# Autodesk Inventor assembly: RobotTable
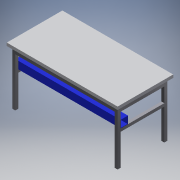
[picture p0: Inventor's stored thumbnail of the model, 180x180]
Saved by Autodesk Inventor 2017 (Build 210142000, 142)
## iProperties
Created: 2018-08-24
Part Number: RobotTable
Document SubType Name: Assembly
Designer: emmacarlisle
Author: emmacarlisle
## Documents named in this file (4)
- \\Mac\Home\Documents\RobotTable.iam
- \\Mac\Home\Documents\bottomtable.ipt
- \\Mac\Home\Documents\toptable.ipt
- \\Mac\Home\Documents\bluethingfortable.ipt
## Components (3 placed, 3 different names)
1. bottomtable:1 — Mate:1, Flush:1, Flush:2, Mate:2, Mate:3, Flush:3
2. toptable:1 — Mate:1, Flush:1, Flush:2
3. bluethingfortable:1 — Mate:2, Mate:3, Flush:3
## Relationships (6: Mate 3, Flush 3)
- Mate:1: bottomtable:1 ↔ toptable:1
- Flush:1: bottomtable:1 ↔ toptable:1
- Flush:2: bottomtable:1 ↔ toptable:1
- Mate:2: bottomtable:1 ↔ bluethingfortable:1
- Mate:3: bottomtable:1 ↔ bluethingfortable:1
- Flush:3: bottomtable:1 ↔ bluethingfortable:1
